# Autodesk Inventor assembly: bumper test
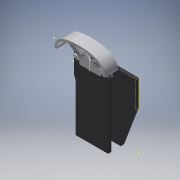
[picture p0: Inventor's stored thumbnail of the model, 180x180]
Saved by Autodesk Inventor 2016 (Build 200138000, 138)
## iProperties
Created: 2015-09-30
Part Number: bumper test
Document SubType Name: Assembly
Designer: Jesse Stevenson
Author: Jesse Stevenson
## Documents named in this file (7)
- C:\Users\Jesse Stevenson\Desktop\E-121-Design\bumper test.iam
- C:\Users\Jesse Stevenson\Desktop\E-121-Design\top.ipt
- C:\Users\Jesse Stevenson\Desktop\E-121-Design\bottom.ipt
- C:\Users\Jesse Stevenson\Desktop\E-121-Design\Microswitch_-_Omron_D2SW-P2L2T.iam
- C:\Users\Jesse Stevenson\Desktop\E-121-Design\bumper lever support.ipt
- C:\Users\Jesse Stevenson\Desktop\E-121-Design\lever2.ipt
- C:\Users\Jesse Stevenson\Desktop\E-121-Design\bumper.ipt
## Components (8 placed, 6 different names)
1. top:1 — Flush:1, Mate:1, Mate:2
2. bottom:1 — Flush:1, Mate:1, Mate:3, Angle:1, Mate:20, Angle:2, Mate:21
3. Microswitch_-_Omron_D2SW-P2L2T:1 [sub-assembly] — Flush:2, Mate:17, Flush:3
4. Microswitch_-_Omron_D2SW-P2L2T:2 [sub-assembly] — Flush:2, Mate:16, Angle:1, Flush:3
5. bumper lever support:1 — Mate:20, Angle:2, Mate:21, Mate:22, Mate:23, Mate:24
6. bumper:1 — Mate:8, Mate:9, Mate:11, Mate:15
7. lever2:1 — Mate:11, Mate:15, Mate:16, Mate:23
8. lever2:2 — Mate:8, Mate:9, Mate:17, Mate:22, Mate:24
## Relationships (20: Mate 15, Flush 3, Angle 2)
- Flush:1: top:1 ↔ bottom:1
- Mate:1 (18.923 mm): top:1 ↔ bottom:1
- Mate:2: top:1
- Mate:3: bottom:1
- Mate:4 (25.273 mm)
- Flush:2: Microswitch_-_Omron_D2SW-P2L2T:1 ↔ Microswitch_-_Omron_D2SW-P2L2T:2
- Mate:8: bumper:1 ↔ lever2:2
- Mate:9: bumper:1 ↔ lever2:2
- Mate:11: bumper:1 ↔ lever2:1
- Mate:15: bumper:1 ↔ lever2:1
- Mate:16 (-1.27 mm): Microswitch_-_Omron_D2SW-P2L2T:2 ↔ lever2:1
- Mate:17 (-1.27 mm): Microswitch_-_Omron_D2SW-P2L2T:1 ↔ lever2:2
- Angle:1 (0 deg): bottom:1 ↔ Microswitch_-_Omron_D2SW-P2L2T:2
- Mate:20: bottom:1 ↔ bumper lever support:1
- Angle:2 (0 deg): bottom:1 ↔ bumper lever support:1
- Mate:21: bottom:1 ↔ bumper lever support:1
- Mate:22: bumper lever support:1 ↔ lever2:2
- Mate:23: bumper lever support:1 ↔ lever2:1
- Mate:24: bumper lever support:1 ↔ lever2:2
- Flush:3: Microswitch_-_Omron_D2SW-P2L2T:1 ↔ Microswitch_-_Omron_D2SW-P2L2T:2
